# Autodesk Inventor assembly: leg_B_12
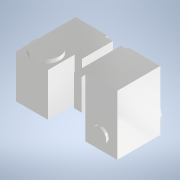
[picture p0: Inventor's stored thumbnail of the model, 180x180]
Saved by Autodesk Inventor 2020.2 (Build 242310000, 310)
## iProperties
Created: 2020-09-17
Part Number: leg_B_12
Document SubType Name: Assembly
Designer: mazzo
Author: mazzo
## Documents named in this file (2)
- D:\Documenti\università\Progetto Meccanica dei Robot\assembled in urdf\leg_B_12.iam
- D:\Documenti\università\Progetto Meccanica dei Robot\meccanica\parti autodesk\V5\Motore2.ipt
## Components (2 placed, 1 different names)
1. Motore2:1 — Coincidente:1, Allineato:1, Angolo:1, Cilindrico:1, Cilindrico:2, Coincidente:2
2. Motore2:2 — Cilindrico:1, Cilindrico:2, Coincidente:2
## Relationships (6: Mate 2, CylindricalJoint 2, Flush 1, Angle 1)
- Coincidente:1 [Mate]: Motore2:1
- Allineato:1 [Flush]: Motore2:1
- Angolo:1 [Angle] (270 deg): Motore2:1
- Cilindrico:1 [CylindricalJoint]: Motore2:1 ↔ Motore2:2
- Cilindrico:2 [CylindricalJoint]: Motore2:1 ↔ Motore2:2
- Coincidente:2 [Mate]: Motore2:1 ↔ Motore2:2
